# Autodesk Inventor assembly: Large_drone_rotor_arm_assembly
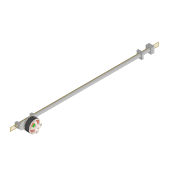
[picture p0: Inventor's stored thumbnail of the model, 180x180]
Saved by Autodesk Inventor 2022 (Build 260153000, 153)
## iProperties
Created: 2022-04-28
Part Number: Large_drone_rotor_arm_assembly
Document SubType Name: Assembly
Designer: dell
Mass: 208.262 g
Surface Area: 351.918 cm^2
Volume: 38.8265 cm^3
Density: 5.36391 g/cm^3
Author: dell
## Documents named in this file (8)
- D:\xxxx\Uni\Part IV\MECHENG_700\Part_IV_project_CAD\Bird_skeleton_prototypes\Wing_drone_V1\Large_drone_rotor_arm_assembly.iam
- D:\xxxx\Uni\Part IV\MECHENG_700\Part_IV_project_CAD\Bird_skeleton_prototypes\Wing_drone_V1\Tube_mount.ipt
- D:\xxxx\Uni\Part IV\MECHENG_700\Part_IV_project_CAD\Bird_skeleton_prototypes\Wing_drone_V1\Tube_adaptor.ipt
- D:\xxxx\Uni\Part IV\MECHENG_700\Part_IV_project_CAD\Bird_skeleton_prototypes\Wing_drone_V1\Tube_mount_centering.ipt
- D:\xxxx\Uni\Part IV\MECHENG_700\Part_IV_project_CAD\Bird_skeleton_prototypes\Wing_drone_V1\Tube_adaptor_2.ipt
- D:\xxxx\Uni\Part IV\MECHENG_700\Part_IV_project_CAD\Bird_skeleton_prototypes\Wing_drone_V1\CF_tube_12mm_large.ipt
- D:\xxxx\Uni\Part IV\MECHENG_700\Part_IV_project_CAD\Bird_skeleton_prototypes\Wing_drone_V1\Motor_mount_plate_large.ipt
- D:\xxxx\Uni\Part IV\MECHENG_700\Part_IV_project_CAD\Bird_skeleton_prototypes\Wing_drone_V1\MN4014\MN4014MotorAssembly.iam
## Components (11 placed, 7 different names)
1. Tube_mount:1 — Mate:24, Mate:36
2. Tube_mount:3 — Mate:24, Mate:35, Angle:7, Mate:37
3. Tube_adaptor:1 — Mate:43, Mate:45, Mate:47, Mate:48
4. Tube_adaptor:2 — Mate:42, Mate:44, Mate:46, Mate:52
5. Tube_mount_centering:1 — Mate:31, Mate:32, Angle:7
6. Tube_mount_centering:2 — Mate:33, Mate:34
7. Tube_adaptor_2:1 — Mate:40, Mate:41
8. Tube_adaptor_2:2 — Mate:38, Mate:39
9. CF_tube_12mm_large:1 — Mate:31, Mate:32, Mate:33, Mate:34, Mate:35, Mate:36, Mate:37, Mate:38, Mate:39, Mate:40, Mate:41, Mate:42, Mate:43, Mate:44, Mate:45, Mate:47
10. Motor_mount_plate_large:1 — Mate:46, Mate:48, Mate:49, Mate:50, Mate:51, Mate:52
11. MN4014MotorAssembly:2 [sub-assembly] — Mate:49, Mate:50, Mate:51
## Relationships (24: Mate 23, Angle 1)
- Mate:24: Tube_mount:1 ↔ Tube_mount:3
- Mate:31: Tube_mount_centering:1 ↔ CF_tube_12mm_large:1
- Mate:32: Tube_mount_centering:1 ↔ CF_tube_12mm_large:1
- Mate:33: Tube_mount_centering:2 ↔ CF_tube_12mm_large:1
- Mate:34: Tube_mount_centering:2 ↔ CF_tube_12mm_large:1
- Mate:35: Tube_mount:3 ↔ CF_tube_12mm_large:1
- Mate:36: Tube_mount:1 ↔ CF_tube_12mm_large:1
- Angle:7 (0 deg): Tube_mount:3 ↔ Tube_mount_centering:1
- Mate:37 (-43.5 mm): Tube_mount:3 ↔ CF_tube_12mm_large:1
- Mate:38: Tube_adaptor_2:2 ↔ CF_tube_12mm_large:1
- Mate:39: Tube_adaptor_2:2 ↔ CF_tube_12mm_large:1
- Mate:40: Tube_adaptor_2:1 ↔ CF_tube_12mm_large:1
- Mate:41: Tube_adaptor_2:1 ↔ CF_tube_12mm_large:1
- Mate:42: Tube_adaptor:2 ↔ CF_tube_12mm_large:1
- Mate:43: Tube_adaptor:1 ↔ CF_tube_12mm_large:1
- Mate:44: Tube_adaptor:2 ↔ CF_tube_12mm_large:1
- Mate:45: Tube_adaptor:1 ↔ CF_tube_12mm_large:1
- Mate:46: Tube_adaptor:2 ↔ Motor_mount_plate_large:1
- Mate:47: Tube_adaptor:1 ↔ CF_tube_12mm_large:1
- Mate:48: Tube_adaptor:1 ↔ Motor_mount_plate_large:1
- Mate:49: Motor_mount_plate_large:1 ↔ MN4014MotorAssembly:2
- Mate:50: Motor_mount_plate_large:1 ↔ MN4014MotorAssembly:2
- Mate:51: Motor_mount_plate_large:1 ↔ MN4014MotorAssembly:2
- Mate:52: Tube_adaptor:2 ↔ Motor_mount_plate_large:1
